# Autodesk Inventor assembly: FirstIntakes
(part 2 of 3)
- [Mate]: 1_2” Hex Bore Plastic VersaHub v2 (217-8079):20 ↔ #8-32 Nylock Nut (275-1027):49
- [Angle] (0 deg): 1_2” Hex Bore Plastic VersaHub v2 (217-8079):20 ↔ #8-32 Nylock Nut (275-1027):54
- [Angle] (0 deg): 1_2” Hex Bore Plastic VersaHub v2 (217-8079):20 ↔ #8-32 Nylock Nut (275-1027):49
- [Angle] (0 deg): 1_2” Hex Bore Plastic VersaHub v2 (217-8079):20 ↔ #8-32 Nylock Nut (275-1027):53
- [Angle] (0 deg): 1_2” Hex Bore Plastic VersaHub v2 (217-8079):20 ↔ #8-32 Nylock Nut (275-1027):50
- [Angle] (0 deg): 1_2” Hex Bore Plastic VersaHub v2 (217-8079):20 ↔ #8-32 Nylock Nut (275-1027):52
- [Angle] (0 deg): 1_2” Hex Bore Plastic VersaHub v2 (217-8079):20 ↔ #8-32 Nylock Nut (275-1027):51
- [Mate]: 1_2” Hex Bore Plastic VersaHub v2 (217-8079):19 ↔ 1_4 Acetal Spacer - 1_2 Hex (217-2758):10
- [Angle] (0 deg): 1_2” Hex Bore Plastic VersaHub v2 (217-8079):19 ↔ 1_4 Acetal Spacer - 1_2 Hex (217-2758):10
- [Mate]: 1_2” Hex Bore Plastic VersaHub v2 (217-8079):19 ↔ 1_4 Acetal Spacer - 1_2 Hex (217-2758):10
- Mate:406: 5 Straight Flex Wheel (60A) (217-6455):4 ↔ 5 Straight Flex Wheel (60A) (217-6455):10
- Mate:407: 5 Straight Flex Wheel (60A) (217-6455):4 ↔ 5 Straight Flex Wheel (60A) (217-6455):11
- Mate:410: 5 Straight Flex Wheel (60A) (217-6455):5 ↔ 5 Straight Flex Wheel (60A) (217-6455):6
- [Mate]: 5 Straight Flex Wheel (60A) (217-6455):12 ↔ 1_2” Hex Bore Plastic VersaHub v2 (217-8079):22
- [Mate]: 5 Straight Flex Wheel (60A) (217-6455):12 ↔ 1_2” Hex Bore Plastic VersaHub v2 (217-8079):22
- [Mate]: 5 Straight Flex Wheel (60A) (217-6455):12 ↔ 1_2” Hex Bore Plastic VersaHub v2 (217-8079):22
- [Mate]: 5 Straight Flex Wheel (60A) (217-6455):12 ↔ 1_2” Hex Bore Plastic VersaHub v2 (217-8079):21
- [Mate]: 5 Straight Flex Wheel (60A) (217-6455):12 ↔ 1_2” Hex Bore Plastic VersaHub v2 (217-8079):21
- [Mate]: 5 Straight Flex Wheel (60A) (217-6455):12 ↔ 1_2” Hex Bore Plastic VersaHub v2 (217-8079):21
- [Mate]: 1_2” Hex Bore Plastic VersaHub v2 (217-8079):21 ↔ #8-32 x 2.000 Star Drive Screw (276-8015):57
- [Mate]: 1_2” Hex Bore Plastic VersaHub v2 (217-8079):21 ↔ #8-32 x 2.000 Star Drive Screw (276-8015):58
- [Mate]: 1_2” Hex Bore Plastic VersaHub v2 (217-8079):21 ↔ #8-32 x 2.000 Star Drive Screw (276-8015):60
- [Mate]: 1_2” Hex Bore Plastic VersaHub v2 (217-8079):21 ↔ #8-32 x 2.000 Star Drive Screw (276-8015):55
- [Mate]: 1_2” Hex Bore Plastic VersaHub v2 (217-8079):21 ↔ #8-32 x 2.000 Star Drive Screw (276-8015):56
- [Mate]: 1_2” Hex Bore Plastic VersaHub v2 (217-8079):21 ↔ #8-32 x 2.000 Star Drive Screw (276-8015):59
- [Mate]: 1_2” Hex Bore Plastic VersaHub v2 (217-8079):21 ↔ #8-32 x 2.000 Star Drive Screw (276-8015):56
- [Mate]: 1_2” Hex Bore Plastic VersaHub v2 (217-8079):21 ↔ #8-32 x 2.000 Star Drive Screw (276-8015):58
- [Mate]: 1_2” Hex Bore Plastic VersaHub v2 (217-8079):21 ↔ #8-32 x 2.000 Star Drive Screw (276-8015):57
- [Mate]: 1_2” Hex Bore Plastic VersaHub v2 (217-8079):21 ↔ #8-32 x 2.000 Star Drive Screw (276-8015):59
- [Mate]: 1_2” Hex Bore Plastic VersaHub v2 (217-8079):21 ↔ #8-32 x 2.000 Star Drive Screw (276-8015):55
- [Mate]: 1_2” Hex Bore Plastic VersaHub v2 (217-8079):21 ↔ #8-32 x 2.000 Star Drive Screw (276-8015):60
- [Mate]: #8-32 x 2.000 Star Drive Screw (276-8015):57 ↔ #8-32 Nylock Nut (275-1027):60
- [Mate]: #8-32 x 2.000 Star Drive Screw (276-8015):60 ↔ #8-32 Nylock Nut (275-1027):55
- [Mate]: #8-32 x 2.000 Star Drive Screw (276-8015):55 ↔ #8-32 Nylock Nut (275-1027):59
- [Mate]: #8-32 x 2.000 Star Drive Screw (276-8015):59 ↔ #8-32 Nylock Nut (275-1027):56
- [Mate]: #8-32 x 2.000 Star Drive Screw (276-8015):56 ↔ #8-32 Nylock Nut (275-1027):58
- [Mate]: #8-32 x 2.000 Star Drive Screw (276-8015):58 ↔ #8-32 Nylock Nut (275-1027):57
- [Mate]: 1_2” Hex Bore Plastic VersaHub v2 (217-8079):22 ↔ #8-32 Nylock Nut (275-1027):60
- [Mate]: 1_2” Hex Bore Plastic VersaHub v2 (217-8079):22 ↔ #8-32 Nylock Nut (275-1027):57
- [Mate]: 1_2” Hex Bore Plastic VersaHub v2 (217-8079):22 ↔ #8-32 Nylock Nut (275-1027):58
- [Mate]: 1_2” Hex Bore Plastic VersaHub v2 (217-8079):22 ↔ #8-32 Nylock Nut (275-1027):56
- [Mate]: 1_2” Hex Bore Plastic VersaHub v2 (217-8079):22 ↔ #8-32 Nylock Nut (275-1027):59
- [Mate]: 1_2” Hex Bore Plastic VersaHub v2 (217-8079):22 ↔ #8-32 Nylock Nut (275-1027):55
- [Angle] (0 deg): 1_2” Hex Bore Plastic VersaHub v2 (217-8079):22 ↔ #8-32 Nylock Nut (275-1027):60
- [Angle] (0 deg): 1_2” Hex Bore Plastic VersaHub v2 (217-8079):22 ↔ #8-32 Nylock Nut (275-1027):55
- [Angle] (0 deg): 1_2” Hex Bore Plastic VersaHub v2 (217-8079):22 ↔ #8-32 Nylock Nut (275-1027):59
- [Angle] (0 deg): 1_2” Hex Bore Plastic VersaHub v2 (217-8079):22 ↔ #8-32 Nylock Nut (275-1027):56
- [Angle] (0 deg): 1_2” Hex Bore Plastic VersaHub v2 (217-8079):22 ↔ #8-32 Nylock Nut (275-1027):58
- [Angle] (0 deg): 1_2” Hex Bore Plastic VersaHub v2 (217-8079):22 ↔ #8-32 Nylock Nut (275-1027):57
- Mate:444: 5 Straight Flex Wheel (60A) (217-6455):5 ↔ 5 Straight Flex Wheel (60A) (217-6455):12
- Mate:446: 1_2” Hex Bore Plastic VersaHub v2 (217-8079):22 ↔ 1_2 Acetal Spacer - 1_2 Hex (217-2758):3
- Angle:132 (0 deg): 1_2” Hex Bore Plastic VersaHub v2 (217-8079):22 ↔ 1_2 Acetal Spacer - 1_2 Hex (217-2758):3
- Mate:447: 1_2” Hex Bore Plastic VersaHub v2 (217-8079):22 ↔ 1_2 Acetal Spacer - 1_2 Hex (217-2758):3
- Flush:1: 5 Straight Flex Wheel (60A) (217-6455):4 ↔ 5 Straight Flex Wheel (60A) (217-6455):5
- Flush:2: 5 Straight Flex Wheel (60A) (217-6455):3 ↔ 5 Straight Flex Wheel (60A) (217-6455):4
- Mate:448: 13.75mm (1_2 ThunderHex ID) x 1.125 OD x 0.313 WD (Flanged Bearing) (217-4006):2 ↔ 5 Straight Flex Wheel (60A) (217-6455):4
- Angle:133 (0 deg): 1 x 1 x 0.040 x 14 Intake Pre-Drilled VersaFrame Aluminum Tube Stock Cut Modified (217-3426):1 ↔ 24T x 9mm Wide Double Flange Aluminum Pulley (HTD 5mm, 1_2” Hex Bore) (217-3227):8
- Angle:134 (0 deg): 1 x 1 x 0.040 x 14 Intake Pre-Drilled VersaFrame Aluminum Tube Stock Cut Modified (217-3426):1 ↔ 24T x 9mm Wide Double Flange Aluminum Pulley (HTD 5mm, 1_2” Hex Bore) (217-3227):6
- Angle:135 (0 deg): 1 x 1 x 0.040 x 14 Intake Pre-Drilled VersaFrame Aluminum Tube Stock Cut Modified (217-3426):1 ↔ 1_4 Acetal Spacer - 1_2 Hex (217-2758):13
- Angle:136 (0 deg): 1 x 1 x 0.040 x 14 Intake Pre-Drilled VersaFrame Aluminum Tube Stock Cut Modified (217-3426):1 ↔ 1_2” Hex Bore Plastic VersaHub v2 (217-8079):20
- Angle:139 (0 deg): 24T x 9mm Wide Double Flange Aluminum Pulley (HTD 5mm, 1_2” Hex Bore) (217-3227):8 ↔ 1_2 Acetal Spacer - 1_2 Hex (217-2758):3
- Angle:140 (0 deg): 24T x 9mm Wide Double Flange Aluminum Pulley (HTD 5mm, 1_2” Hex Bore) (217-3227):8 ↔ 1_2 Acetal Spacer - 1_2 Hex (217-2758):3
- Flush:4: 5 Straight Flex Wheel (60A) (217-6455):6 ↔ 5 Straight Flex Wheel (60A) (217-6455):11
- Mate:452: 24T x 9mm Wide Double Flange Aluminum Pulley (HTD 5mm, 1_2” Hex Bore) (217-3227):6 ↔ 1_4 Acetal Spacer - 1_2 Hex (217-2758):10
- Mate:453: 5 Straight Flex Wheel (60A) (217-6455):11 ↔ 80T x 9mm Wide Timing Belt (HTD 5mm)(217-3456):2
- Mate:454: 5 Straight Flex Wheel (60A) (217-6455):11 ↔ 80T x 9mm Wide Timing Belt (HTD 5mm)(217-3456):1
- Mate:455: 5 Straight Flex Wheel (60A) (217-6455):3 ↔ 80T x 9mm Wide Timing Belt (HTD 5mm)(217-3456):2
- Mate:456: 5 Straight Flex Wheel (60A) (217-6455):6 ↔ 80T x 9mm Wide Timing Belt (HTD 5mm)(217-3456):1
- Flush:5: 24T x 9mm Wide Double Flange Aluminum Pulley (HTD 5mm, 1_2” Hex Bore) (217-3227):3 ↔ 80T x 9mm Wide Timing Belt (HTD 5mm)(217-3456):2
- Flush:6: 24T x 9mm Wide Double Flange Aluminum Pulley (HTD 5mm, 1_2” Hex Bore) (217-3227):6 ↔ 80T x 9mm Wide Timing Belt (HTD 5mm)(217-3456):1
- Mate:462: 1_2” Hex Bore Plastic VersaHub v2 (217-8079):17 ↔ Clamping Shaft Collar - 1_2 Hex ID (217-2737):4
- Angle:181 (0 deg): 1_2” Hex Bore Plastic VersaHub v2 (217-8079):17 ↔ Clamping Shaft Collar - 1_2 Hex ID (217-2737):4
- Angle:182 (0 deg): Clamping Shaft Collar - 1_2 Hex ID (217-2737):4 ↔ Clamping Shaft Collar - 1_2 Hex ID (217-2737):6
- Mate:463: 1_4 Acetal Spacer - 1_2 Hex (217-2758):12 ↔ Clamping Shaft Collar - 1_2 Hex ID (217-2737):6
- Mate:464: 1_2” Hex Bore Plastic VersaHub v2 (217-8079):20 ↔ Clamping Shaft Collar - 1_2 Hex ID (217-2737):3
- Mate:465: 1_2” Hex Bore Plastic VersaHub v2 (217-8079):20 ↔ Clamping Shaft Collar - 1_2 Hex ID (217-2737):3
- Angle:183 (0 deg): 1_2” Hex Bore Plastic VersaHub v2 (217-8079):20 ↔ Clamping Shaft Collar - 1_2 Hex ID (217-2737):3
- Angle:185 (0 deg): 1_2” Hex Bore Plastic VersaHub v2 (217-8079):4 ↔ Clamping Shaft Collar - 1_2 Hex ID (217-2737):9
- Angle:186 (0 deg): 1_2” Hex Bore Plastic VersaHub v2 (217-8079):4 ↔ Clamping Shaft Collar - 1_2 Hex ID (217-2737):9
- Mate:467: 1_2” Hex Bore Plastic VersaHub v2 (217-8079):4 ↔ Clamping Shaft Collar - 1_2 Hex ID (217-2737):9
- Mate:468: 1_2” Hex Bore Plastic VersaHub v2 (217-8079):4 ↔ Clamping Shaft Collar - 1_2 Hex ID (217-2737):9
- Mate:470: 24T x 9mm Wide Double Flange Aluminum Pulley (HTD 5mm, 1_2” Hex Bore) (217-3227):3 ↔ Clamping Shaft Collar - 1_2 Hex ID (217-2737):7
- Mate:471: 24T x 9mm Wide Double Flange Aluminum Pulley (HTD 5mm, 1_2” Hex Bore) (217-3227):3 ↔ Clamping Shaft Collar - 1_2 Hex ID (217-2737):10
- Mate:472: 24T x 9mm Wide Double Flange Aluminum Pulley (HTD 5mm, 1_2” Hex Bore) (217-3227):3 ↔ Clamping Shaft Collar - 1_2 Hex ID (217-2737):10
- Angle:188 (0 deg): 24T x 9mm Wide Double Flange Aluminum Pulley (HTD 5mm, 1_2” Hex Bore) (217-3227):3 ↔ Clamping Shaft Collar - 1_2 Hex ID (217-2737):10
- Angle:189 (0 deg): Clamping Shaft Collar - 1_2 Hex ID (217-2737):7 ↔ Clamping Shaft Collar - 1_2 Hex ID (217-2737):10
- Mate:474: 1_2” Hex Bore Plastic VersaHub v2 (217-8079):17 ↔ 1_4 Acetal Spacer - 1_2 Hex (217-2758):13
- Mate:475: 1_2” Hex Bore Plastic VersaHub v2 (217-8079):18 ↔ Clamping Shaft Collar - 1_2 Hex ID (217-2737):4
- Flush:11: 5 Straight Flex Wheel (60A) (217-6455):10 ↔ 5 Straight Flex Wheel (60A) (217-6455):12
- Mate:476: 24T x 9mm Wide Double Flange Aluminum Pulley (HTD 5mm, 1_2” Hex Bore) (217-3227):5 ↔ 1_4 Acetal Spacer - 1_2 Hex (217-2758):13
- Mate:477: 5 Straight Flex Wheel (60A) (217-6455):4 ↔ 5 Straight Flex Wheel (60A) (217-6455):10
- Mate:486: 1_2 Acetal Spacer - 1_2 Hex (217-2758):3 ↔ 1_16 Acetal Spacer - 1_2 Hex (217-2758):2
- Angle:199 (0 deg): 1_2 Acetal Spacer - 1_2 Hex (217-2758):3 ↔ 1_16 Acetal Spacer - 1_2 Hex (217-2758):2
- Mate:487: 1_2 Acetal Spacer - 1_2 Hex (217-2758):4 ↔ 1_16 Acetal Spacer - 1_2 Hex (217-2758):2
- Mate:494: 1 x 1 x 0.040 x 14 Intake Pre-Drilled VersaFrame Aluminum Tube Stock Cut Modified (217-3426):1 ↔ #8-32 x 1.500 Star Drive Screw (276-4998):1
- Mate:495: 1 x 1 x 0.040 x 14 Intake Pre-Drilled VersaFrame Aluminum Tube Stock Cut Modified (217-3426):1 ↔ #8-32 x 1.500 Star Drive Screw (276-4998):2
- Mate:496: 1 x 1 x 0.040 x 14 Intake Pre-Drilled VersaFrame Aluminum Tube Stock Cut Modified (217-3426):1 ↔ #8-32 x 1.500 Star Drive Screw (276-4998):3
- Mate:497: 1 x 1 x 0.040 x 14 Intake Pre-Drilled VersaFrame Aluminum Tube Stock Cut Modified (217-3426):1 ↔ #8-32 x 1.500 Star Drive Screw (276-4998):4
- Mate:498: 1 x 1 x 0.040 x 14 Intake Pre-Drilled VersaFrame Aluminum Tube Stock Cut Modified (217-3426):1 ↔ #8-32 x 1.500 Star Drive Screw (276-4998):5
- Mate:499: 1 x 1 x 0.040 x 14 Intake Pre-Drilled VersaFrame Aluminum Tube Stock Cut Modified (217-3426):1 ↔ #8-32 x 1.500 Star Drive Screw (276-4998):7
- Mate:500: 1 x 1 x 0.040 x 14 Intake Pre-Drilled VersaFrame Aluminum Tube Stock Cut Modified (217-3426):1 ↔ #8-32 x 1.500 Star Drive Screw (276-4998):6
- Mate:501: 1 x 1 x 0.040 x 14 Intake Pre-Drilled VersaFrame Aluminum Tube Stock Cut Modified (217-3426):1 ↔ #8-32 x 1.500 Star Drive Screw (276-4998):8
- Mate:505: 1 x 1 x 0.040 x 14 Intake Pre-Drilled VersaFrame Aluminum Tube Stock Cut Modified (217-3426):1 ↔ #8-32 x 1.500 Star Drive Screw (276-4998):4
- Mate:506: 1 x 1 x 0.040 x 14 Intake Pre-Drilled VersaFrame Aluminum Tube Stock Cut Modified (217-3426):1 ↔ #8-32 x 1.500 Star Drive Screw (276-4998):5
- Mate:510: #8-32 x 1.500 Star Drive Screw (276-4998):1 ↔ #8-32 Nylock Nut (275-1027):65
- Mate:511: #8-32 x 1.500 Star Drive Screw (276-4998):2 ↔ #8-32 Nylock Nut (275-1027):63
- Mate:512: #8-32 x 1.500 Star Drive Screw (276-4998):3 ↔ #8-32 Nylock Nut (275-1027):64
- Mate:513: #8-32 x 1.500 Star Drive Screw (276-4998):5 ↔ #8-32 Nylock Nut (275-1027):62
- Mate:514: #8-32 x 1.500 Star Drive Screw (276-4998):4 ↔ #8-32 Nylock Nut (275-1027):61
- Mate:515: #8-32 x 1.500 Star Drive Screw (276-4998):8 ↔ #8-32 Nylock Nut (275-1027):66
- Mate:516: #8-32 x 1.500 Star Drive Screw (276-4998):6 ↔ #8-32 Nylock Nut (275-1027):67
- Mate:517: #8-32 x 1.500 Star Drive Screw (276-4998):7 ↔ #8-32 Nylock Nut (275-1027):68
- Mate:521: VersaFrame Side Bearing Gusset (217-3553):2 ↔ #8-32 Nylock Nut (275-1027):61
- Mate:522: VersaFrame Side Bearing Gusset (217-3553):2 ↔ #8-32 Nylock Nut (275-1027):62
- Mate:523: VersaFrame Side Bearing Gusset (217-3553):3 ↔ #8-32 Nylock Nut (275-1027):65
- Mate:524: VersaFrame Side Bearing Gusset (217-3553):3 ↔ #8-32 Nylock Nut (275-1027):63
- Mate:525: VersaFrame Side Bearing Gusset (217-3553):3 ↔ #8-32 Nylock Nut (275-1027):64
- Angle:203 (0 deg): 1 x 1 x 0.040 x 14 Intake Pre-Drilled VersaFrame Aluminum Tube Stock Cut Modified (217-3426):1 ↔ #8-32 Nylock Nut (275-1027):66
- Angle:204 (0 deg): 1 x 1 x 0.040 x 14 Intake Pre-Drilled VersaFrame Aluminum Tube Stock Cut Modified (217-3426):1 ↔ #8-32 Nylock Nut (275-1027):67
- Angle:205 (0 deg): 1 x 1 x 0.040 x 14 Intake Pre-Drilled VersaFrame Aluminum Tube Stock Cut Modified (217-3426):1 ↔ #8-32 Nylock Nut (275-1027):68
- Angle:206 (0 deg): 1 x 1 x 0.040 x 14 Intake Pre-Drilled VersaFrame Aluminum Tube Stock Cut Modified (217-3426):1 ↔ #8-32 Nylock Nut (275-1027):61
- Angle:207 (0 deg): 1 x 1 x 0.040 x 14 Intake Pre-Drilled VersaFrame Aluminum Tube Stock Cut Modified (217-3426):1 ↔ #8-32 Nylock Nut (275-1027):62
- Angle:208 (0 deg): 1 x 1 x 0.040 x 14 Intake Pre-Drilled VersaFrame Aluminum Tube Stock Cut Modified (217-3426):1 ↔ #8-32 Nylock Nut (275-1027):64
- Angle:209 (0 deg): 1 x 1 x 0.040 x 14 Intake Pre-Drilled VersaFrame Aluminum Tube Stock Cut Modified (217-3426):1 ↔ #8-32 Nylock Nut (275-1027):63
- Angle:210 (0 deg): 1 x 1 x 0.040 x 14 Intake Pre-Drilled VersaFrame Aluminum Tube Stock Cut Modified (217-3426):1 ↔ #8-32 Nylock Nut (275-1027):65
- Angle:211 (0 deg): 1 x 1 x 0.040 x 14 Intake Pre-Drilled VersaFrame Aluminum Tube Stock Cut Modified (217-3426):1 ↔ #8-32 x 1.500 Star Drive Screw (276-4998):1
- Angle:212 (0 deg): 1 x 1 x 0.040 x 14 Intake Pre-Drilled VersaFrame Aluminum Tube Stock Cut Modified (217-3426):1 ↔ #8-32 x 1.500 Star Drive Screw (276-4998):8
- Angle:213 (0 deg): 1 x 1 x 0.040 x 14 Intake Pre-Drilled VersaFrame Aluminum Tube Stock Cut Modified (217-3426):1 ↔ #8-32 x 1.500 Star Drive Screw (276-4998):7
- Angle:214 (0 deg): 1 x 1 x 0.040 x 14 Intake Pre-Drilled VersaFrame Aluminum Tube Stock Cut Modified (217-3426):1 ↔ #8-32 x 1.500 Star Drive Screw (276-4998):6
- Angle:215 (0 deg): 1 x 1 x 0.040 x 14 Intake Pre-Drilled VersaFrame Aluminum Tube Stock Cut Modified (217-3426):1 ↔ #8-32 x 1.500 Star Drive Screw (276-4998):5
- Angle:216 (0 deg): 1 x 1 x 0.040 x 14 Intake Pre-Drilled VersaFrame Aluminum Tube Stock Cut Modified (217-3426):1 ↔ #8-32 x 1.500 Star Drive Screw (276-4998):4
- Angle:217 (0 deg): 1 x 1 x 0.040 x 14 Intake Pre-Drilled VersaFrame Aluminum Tube Stock Cut Modified (217-3426):1 ↔ #8-32 x 1.500 Star Drive Screw (276-4998):3
- Angle:218 (0 deg): 1 x 1 x 0.040 x 14 Intake Pre-Drilled VersaFrame Aluminum Tube Stock Cut Modified (217-3426):1 ↔ #8-32 x 1.500 Star Drive Screw (276-4998):2
- Mate:526: 13.75mm (1_2 ThunderHex ID) x 1.125 OD x 0.313 WD (Flanged Bearing) (217-4006):2 ↔ Clamping Shaft Collar - 1_2 Hex ID (217-2737):6
- Mate:529: #8-32 Nylock Nut (275-1027):69 ↔ #8-32 x 2.000 Star Drive Screw (276-8015):61
- Mate:530: #8-32 Nylock Nut (275-1027):70 ↔ #8-32 x 2.000 Star Drive Screw (276-8015):63
- Mate:531: #8-32 Nylock Nut (275-1027):71 ↔ #8-32 x 2.000 Star Drive Screw (276-8015):66
- Mate:532: #8-32 Nylock Nut (275-1027):72 ↔ #8-32 x 2.000 Star Drive Screw (276-8015):64
- Mate:533: #8-32 Nylock Nut (275-1027):73 ↔ #8-32 x 2.000 Star Drive Screw (276-8015):65
- Mate:534: #8-32 Nylock Nut (275-1027):80 ↔ #8-32 x 2.000 Star Drive Screw (276-8015):62
- Mate:535: #8-32 Nylock Nut (275-1027):74 ↔ #8-32 x 2.000 Star Drive Screw (276-8015):67
- Mate:536: #8-32 Nylock Nut (275-1027):75 ↔ #8-32 x 2.000 Star Drive Screw (276-8015):68
- Mate:537: #8-32 Nylock Nut (275-1027):79 ↔ #8-32 x 2.000 Star Drive Screw (276-8015):69
- Mate:538: #8-32 Nylock Nut (275-1027):76 ↔ #8-32 x 2.000 Star Drive Screw (276-8015):71
- Mate:539: #8-32 Nylock Nut (275-1027):77 ↔ #8-32 x 2.000 Star Drive Screw (276-8015):70
- Mate:540: #8-32 Nylock Nut (275-1027):78 ↔ #8-32 x 2.000 Star Drive Screw (276-8015):72
- Angle:219 (0 deg): 1_2” Hex Bore Plastic VersaHub v2 (217-8079):6 ↔ #8-32 Nylock Nut (275-1027):70
- Angle:220 (0 deg): 1_2” Hex Bore Plastic VersaHub v2 (217-8079):6 ↔ #8-32 Nylock Nut (275-1027):71
- Angle:221 (0 deg): 1_2” Hex Bore Plastic VersaHub v2 (217-8079):6 ↔ #8-32 Nylock Nut (275-1027):72
- Angle:222 (0 deg): 1_2” Hex Bore Plastic VersaHub v2 (217-8079):6 ↔ #8-32 Nylock Nut (275-1027):73
- Angle:223 (0 deg): 1_2” Hex Bore Plastic VersaHub v2 (217-8079):6 ↔ #8-32 Nylock Nut (275-1027):80
- Angle:224 (0 deg): 1_2” Hex Bore Plastic VersaHub v2 (217-8079):6 ↔ #8-32 Nylock Nut (275-1027):69
- Angle:225 (0 deg): 1_2” Hex Bore Plastic VersaHub v2 (217-8079):8 ↔ #8-32 Nylock Nut (275-1027):78
- Angle:226 (0 deg): 1_2” Hex Bore Plastic VersaHub v2 (217-8079):8 ↔ #8-32 Nylock Nut (275-1027):76
- Angle:227 (0 deg): 1_2” Hex Bore Plastic VersaHub v2 (217-8079):8 ↔ #8-32 Nylock Nut (275-1027):75
- Angle:228 (0 deg): 1_2” Hex Bore Plastic VersaHub v2 (217-8079):8 ↔ #8-32 Nylock Nut (275-1027):74
- Angle:229 (0 deg): 1_2” Hex Bore Plastic VersaHub v2 (217-8079):8 ↔ #8-32 Nylock Nut (275-1027):77
- Angle:230 (0 deg): 1_2” Hex Bore Plastic VersaHub v2 (217-8079):8 ↔ #8-32 Nylock Nut (275-1027):79
- Mate:541: 1_2” Hex Bore Plastic VersaHub v2 (217-8079):8 ↔ #8-32 Nylock Nut (275-1027):74
- Mate:542: 1_2” Hex Bore Plastic VersaHub v2 (217-8079):8 ↔ #8-32 Nylock Nut (275-1027):79
- Mate:543: 1_2” Hex Bore Plastic VersaHub v2 (217-8079):8 ↔ #8-32 Nylock Nut (275-1027):75
- Mate:544: 1_2” Hex Bore Plastic VersaHub v2 (217-8079):8 ↔ #8-32 Nylock Nut (275-1027):77
- Mate:545: 1_2” Hex Bore Plastic VersaHub v2 (217-8079):8 ↔ #8-32 Nylock Nut (275-1027):76
- Mate:546: 1_2” Hex Bore Plastic VersaHub v2 (217-8079):8 ↔ #8-32 Nylock Nut (275-1027):78
- Mate:547: 1_2” Hex Bore Plastic VersaHub v2 (217-8079):6 ↔ #8-32 Nylock Nut (275-1027):73
- Mate:548: 1_2” Hex Bore Plastic VersaHub v2 (217-8079):6 ↔ #8-32 Nylock Nut (275-1027):71
- Mate:550: 1_2” Hex Bore Plastic VersaHub v2 (217-8079):6 ↔ #8-32 Nylock Nut (275-1027):72
- Mate:551: 1_2” Hex Bore Plastic VersaHub v2 (217-8079):6 ↔ #8-32 Nylock Nut (275-1027):80
- Mate:552: 1_2” Hex Bore Plastic VersaHub v2 (217-8079):6 ↔ #8-32 Nylock Nut (275-1027):69
- Mate:553: 1_2” Hex Bore Plastic VersaHub v2 (217-8079):6 ↔ #8-32 Nylock Nut (275-1027):70
- Angle:231 (0 deg): 1_2” Hex Bore Plastic VersaHub v2 (217-8079):21 ↔ Clamping Shaft Collar - 1_2 Hex ID (217-2737):12
- Mate:554: 1_2” Hex Bore Plastic VersaHub v2 (217-8079):21 ↔ Clamping Shaft Collar - 1_2 Hex ID (217-2737):12
- Mate:555: 1_2” Hex Bore Plastic VersaHub v2 (217-8079):21 ↔ Clamping Shaft Collar - 1_2 Hex ID (217-2737):12
- Angle:232 (0 deg): 1_2” Hex Bore Plastic VersaHub v2 (217-8079):10 ↔ Clamping Shaft Collar - 1_2 Hex ID (217-2737):11
- Mate:556: 1_2” Hex Bore Plastic VersaHub v2 (217-8079):10 ↔ Clamping Shaft Collar - 1_2 Hex ID (217-2737):11
- Mate:557: 1_2” Hex Bore Plastic VersaHub v2 (217-8079):10 ↔ Clamping Shaft Collar - 1_2 Hex ID (217-2737):11
- Angle:233 (0 deg): Clamping Shaft Collar - 1_2 Hex ID (217-2737):3 ↔ Clamping Shaft Collar - 1_2 Hex ID (217-2737):11
- Mate:558: 5 Straight Flex Wheel (60A) (217-6455):3
- Flush:560: 5 Straight Flex Wheel (60A) (217-6455):3
- Flush:14: 5 Straight Flex Wheel (60A) (217-6455):3
- [Mate]: VersaFrame Side Bearing Gusset (217-3553):4 ↔ 1 x 1 x 0.040 x 14 Intake Pre-Drilled VersaFrame Aluminum Tube Stock Cut Modified (217-3426):2
- [Mate]: VersaFrame Side Bearing Gusset (217-3553):4 ↔ 1 x 1 x 0.040 x 14 Intake Pre-Drilled VersaFrame Aluminum Tube Stock Cut Modified (217-3426):2
- [Mate]: VersaFrame Side Bearing Gusset (217-3553):5 ↔ 1 x 1 x 0.040 x 14 Intake Pre-Drilled VersaFrame Aluminum Tube Stock Cut Modified (217-3426):2
- [Mate]: VersaFrame Side Bearing Gusset (217-3553):5 ↔ 1 x 1 x 0.040 x 14 Intake Pre-Drilled VersaFrame Aluminum Tube Stock Cut Modified (217-3426):2
- [Mate]: VersaFrame Side Bearing Gusset (217-3553):5 ↔ 1 x 1 x 0.040 x 14 Intake Pre-Drilled VersaFrame Aluminum Tube Stock Cut Modified (217-3426):2
- [Mate]: VersaFrame Side Bearing Gusset (217-3553):4 ↔ 13.75mm (1_2 ThunderHex ID) x 1.125 OD x 0.313 WD (Flanged Bearing) (217-4006):6
- [Mate]: VersaFrame Side Bearing Gusset (217-3553):5 ↔ 13.75mm (1_2 ThunderHex ID) x 1.125 OD x 0.313 WD (Flanged Bearing) (217-4006):5
- [Mate]: VersaFrame Side Bearing Gusset (217-3553):5 ↔ 13.75mm (1_2 ThunderHex ID) x 1.125 OD x 0.313 WD (Flanged Bearing) (217-4006):5
- [Mate]: VersaFrame Side Bearing Gusset (217-3553):4 ↔ 13.75mm (1_2 ThunderHex ID) x 1.125 OD x 0.313 WD (Flanged Bearing) (217-4006):6
- [Angle] (0 deg): 1 x 1 x 0.040 x 14 Intake Pre-Drilled VersaFrame Aluminum Tube Stock Cut Modified (217-3426):2 ↔ 13.75mm (1_2 ThunderHex ID) x 1.125 OD x 0.313 WD (Flanged Bearing) (217-4006):5
- [Angle] (0 deg): 1 x 1 x 0.040 x 14 Intake Pre-Drilled VersaFrame Aluminum Tube Stock Cut Modified (217-3426):2 ↔ 13.75mm (1_2 ThunderHex ID) x 1.125 OD x 0.313 WD (Flanged Bearing) (217-4006):6
- [Mate]: 1 x 1 x 0.040 x 14 Intake Pre-Drilled VersaFrame Aluminum Tube Stock Cut Modified (217-3426):2 ↔ #8-32 x 1.500 Star Drive Screw (276-4998):9
- [Mate]: 1 x 1 x 0.040 x 14 Intake Pre-Drilled VersaFrame Aluminum Tube Stock Cut Modified (217-3426):2 ↔ #8-32 x 1.500 Star Drive Screw (276-4998):10
- [Mate]: 1 x 1 x 0.040 x 14 Intake Pre-Drilled VersaFrame Aluminum Tube Stock Cut Modified (217-3426):2 ↔ #8-32 x 1.500 Star Drive Screw (276-4998):11
- [Mate]: 1 x 1 x 0.040 x 14 Intake Pre-Drilled VersaFrame Aluminum Tube Stock Cut Modified (217-3426):2 ↔ #8-32 x 1.500 Star Drive Screw (276-4998):12
- [Mate]: 1 x 1 x 0.040 x 14 Intake Pre-Drilled VersaFrame Aluminum Tube Stock Cut Modified (217-3426):2 ↔ #8-32 x 1.500 Star Drive Screw (276-4998):13
- [Mate]: 1 x 1 x 0.040 x 14 Intake Pre-Drilled VersaFrame Aluminum Tube Stock Cut Modified (217-3426):2 ↔ #8-32 x 1.500 Star Drive Screw (276-4998):15
- [Mate]: 1 x 1 x 0.040 x 14 Intake Pre-Drilled VersaFrame Aluminum Tube Stock Cut Modified (217-3426):2 ↔ #8-32 x 1.500 Star Drive Screw (276-4998):14
- [Mate]: 1 x 1 x 0.040 x 14 Intake Pre-Drilled VersaFrame Aluminum Tube Stock Cut Modified (217-3426):2 ↔ #8-32 x 1.500 Star Drive Screw (276-4998):16
- Mate:583: Intake Joint Holder Using 1__16 Gray Tinted Polycarbonate Sheet (36 x 72) (217-6627):1 ↔ #8-32 x 1.500 Star Drive Screw (276-4998):16
- Mate:584: Intake Joint Holder Using 1__16 Gray Tinted Polycarbonate Sheet (36 x 72) (217-6627):1 ↔ #8-32 x 1.500 Star Drive Screw (276-4998):14
- Mate:585: Intake Joint Holder Using 1__16 Gray Tinted Polycarbonate Sheet (36 x 72) (217-6627):1 ↔ #8-32 x 1.500 Star Drive Screw (276-4998):15
- [Mate]: 1 x 1 x 0.040 x 14 Intake Pre-Drilled VersaFrame Aluminum Tube Stock Cut Modified (217-3426):2 ↔ #8-32 x 1.500 Star Drive Screw (276-4998):12
- [Mate]: 1 x 1 x 0.040 x 14 Intake Pre-Drilled VersaFrame Aluminum Tube Stock Cut Modified (217-3426):2 ↔ #8-32 x 1.500 Star Drive Screw (276-4998):13
- [Mate]: 1 x 1 x 0.040 x 14 Intake Pre-Drilled VersaFrame Aluminum Tube Stock Cut Modified (217-3426):2 ↔ #8-32 x 1.500 Star Drive Screw (276-4998):10
- Mate:590: Intake VersaFrame VersaPlanetary Side Mount Modified (217-4239):1 ↔ #8-32 x 1.500 Star Drive Screw (276-4998):9
- [Mate]: #8-32 x 1.500 Star Drive Screw (276-4998):9 ↔ #8-32 Nylock Nut (275-1027):85
- [Mate]: #8-32 x 1.500 Star Drive Screw (276-4998):10 ↔ #8-32 Nylock Nut (275-1027):83
- [Mate]: #8-32 x 1.500 Star Drive Screw (276-4998):11 ↔ #8-32 Nylock Nut (275-1027):84
- [Mate]: #8-32 x 1.500 Star Drive Screw (276-4998):13 ↔ #8-32 Nylock Nut (275-1027):82
- [Mate]: #8-32 x 1.500 Star Drive Screw (276-4998):12 ↔ #8-32 Nylock Nut (275-1027):81
- [Mate]: #8-32 x 1.500 Star Drive Screw (276-4998):16 ↔ #8-32 Nylock Nut (275-1027):86
- [Mate]: #8-32 x 1.500 Star Drive Screw (276-4998):14 ↔ #8-32 Nylock Nut (275-1027):87
- [Mate]: #8-32 x 1.500 Star Drive Screw (276-4998):15 ↔ #8-32 Nylock Nut (275-1027):88
- [Mate]: VersaFrame Side Bearing Gusset (217-3553):4 ↔ #8-32 Nylock Nut (275-1027):88
- [Mate]: VersaFrame Side Bearing Gusset (217-3553):4 ↔ #8-32 Nylock Nut (275-1027):87
- [Mate]: VersaFrame Side Bearing Gusset (217-3553):5 ↔ #8-32 Nylock Nut (275-1027):81
- [Mate]: VersaFrame Side Bearing Gusset (217-3553):5 ↔ #8-32 Nylock Nut (275-1027):82
- [Angle] (0 deg): 1 x 1 x 0.040 x 14 Intake Pre-Drilled VersaFrame Aluminum Tube Stock Cut Modified (217-3426):2 ↔ #8-32 Nylock Nut (275-1027):86
- [Angle] (0 deg): 1 x 1 x 0.040 x 14 Intake Pre-Drilled VersaFrame Aluminum Tube Stock Cut Modified (217-3426):2 ↔ #8-32 Nylock Nut (275-1027):87
- [Angle] (0 deg): 1 x 1 x 0.040 x 14 Intake Pre-Drilled VersaFrame Aluminum Tube Stock Cut Modified (217-3426):2 ↔ #8-32 Nylock Nut (275-1027):88
- [Angle] (0 deg): 1 x 1 x 0.040 x 14 Intake Pre-Drilled VersaFrame Aluminum Tube Stock Cut Modified (217-3426):2 ↔ #8-32 Nylock Nut (275-1027):81
- [Angle] (0 deg): 1 x 1 x 0.040 x 14 Intake Pre-Drilled VersaFrame Aluminum Tube Stock Cut Modified (217-3426):2 ↔ #8-32 Nylock Nut (275-1027):82
- [Angle] (0 deg): 1 x 1 x 0.040 x 14 Intake Pre-Drilled VersaFrame Aluminum Tube Stock Cut Modified (217-3426):2 ↔ #8-32 Nylock Nut (275-1027):84
- [Angle] (0 deg): 1 x 1 x 0.040 x 14 Intake Pre-Drilled VersaFrame Aluminum Tube Stock Cut Modified (217-3426):2 ↔ #8-32 Nylock Nut (275-1027):83
- [Angle] (0 deg): 1 x 1 x 0.040 x 14 Intake Pre-Drilled VersaFrame Aluminum Tube Stock Cut Modified (217-3426):2 ↔ #8-32 Nylock Nut (275-1027):85
- [Angle] (0 deg): 1 x 1 x 0.040 x 14 Intake Pre-Drilled VersaFrame Aluminum Tube Stock Cut Modified (217-3426):2 ↔ #8-32 x 1.500 Star Drive Screw (276-4998):9
- [Angle] (0 deg): 1 x 1 x 0.040 x 14 Intake Pre-Drilled VersaFrame Aluminum Tube Stock Cut Modified (217-3426):2 ↔ #8-32 x 1.500 Star Drive Screw (276-4998):16
- [Angle] (0 deg): 1 x 1 x 0.040 x 14 Intake Pre-Drilled VersaFrame Aluminum Tube Stock Cut Modified (217-3426):2 ↔ #8-32 x 1.500 Star Drive Screw (276-4998):15
- [Angle] (0 deg): 1 x 1 x 0.040 x 14 Intake Pre-Drilled VersaFrame Aluminum Tube Stock Cut Modified (217-3426):2 ↔ #8-32 x 1.500 Star Drive Screw (276-4998):14
- [Angle] (0 deg): 1 x 1 x 0.040 x 14 Intake Pre-Drilled VersaFrame Aluminum Tube Stock Cut Modified (217-3426):2 ↔ #8-32 x 1.500 Star Drive Screw (276-4998):13
- [Angle] (0 deg): 1 x 1 x 0.040 x 14 Intake Pre-Drilled VersaFrame Aluminum Tube Stock Cut Modified (217-3426):2 ↔ #8-32 x 1.500 Star Drive Screw (276-4998):12
- [Angle] (0 deg): 1 x 1 x 0.040 x 14 Intake Pre-Drilled VersaFrame Aluminum Tube Stock Cut Modified (217-3426):2 ↔ #8-32 x 1.500 Star Drive Screw (276-4998):11
- [Angle] (0 deg): 1 x 1 x 0.040 x 14 Intake Pre-Drilled VersaFrame Aluminum Tube Stock Cut Modified (217-3426):2 ↔ #8-32 x 1.500 Star Drive Screw (276-4998):10
- [Mate]: 13.75mm (1_2 ThunderHex ID) x 1.125 OD x 0.313 WD (Flanged Bearing) (217-4006):5 ↔ Clamping Shaft Collar - 1_2 Hex ID (217-2737):14
- [Mate]: VersaFrame Side Bearing Gusset (217-3553):4 ↔ #8-32 Nylock Nut (275-1027):86
- Mate:610: 5 Straight Flex Wheel (60A) (217-6455):3 ↔ 13.75mm (1_2 ThunderHex ID) x 1.125 OD x 0.313 WD (Flanged Bearing) (217-4006):6
- Mate:611: 13.75mm (1_2 ThunderHex ID) x 1.125 OD x 0.313 WD (Flanged Bearing) (217-4006):6 ↔ Clamping Shaft Collar - 1_2 Hex ID (217-2737):15
- Angle:255 (0 deg): 1 x 1 x 0.040 x 14 Intake Pre-Drilled VersaFrame Aluminum Tube Stock Cut Modified (217-3426):2 ↔ Clamping Shaft Collar - 1_2 Hex ID (217-2737):15
- Angle:257 (0 deg): 1 x 1 x 0.040 x 14 Intake Pre-Drilled VersaFrame Aluminum Tube Stock Cut Modified (217-3426):2 ↔ Clamping Shaft Collar - 1_2 Hex ID (217-2737):14
- Angle:258 (0 deg): 1 x 1 x 0.040 x 14 Intake Pre-Drilled VersaFrame Aluminum Tube Stock Cut Modified (217-3426):1 ↔ Clamping Shaft Collar - 1_2 Hex ID (217-2737):1
- Mate:614: 1 x 1 x 0.040 x 14 Intake Pre-Drilled VersaFrame Aluminum Tube Stock Cut Modified (217-3426):2 ↔ Intake Joint Holder Using 1__16 Gray Tinted Polycarbonate Sheet (36 x 72) (217-6627):1
- Mate:615: 1 x 1 x 0.040 x 14 Intake Pre-Drilled VersaFrame Aluminum Tube Stock Cut Modified (217-3426):2 ↔ Intake Joint Holder Using 1__16 Gray Tinted Polycarbonate Sheet (36 x 72) (217-6627):1
- Mate:616: 1 x 1 x 0.040 x 14 Intake Pre-Drilled VersaFrame Aluminum Tube Stock Cut Modified (217-3426):2 ↔ Intake Joint Holder Using 1__16 Gray Tinted Polycarbonate Sheet (36 x 72) (217-6627):1
- Mate:617: 13.75mm (1_2 ThunderHex ID) x 1.125 OD x 0.313 WD (Flanged Bearing) (217-4006):6 ↔ Clamping Shaft Collar - 1_2 Hex ID (217-2737):15
- Mate:618: 1 x 1 x 0.040 x 14 Intake Pre-Drilled VersaFrame Aluminum Tube Stock Cut Modified (217-3426):2 ↔ Intake Joint Holder Using 1__16 Gray Tinted Polycarbonate Sheet (36 x 72) (217-6627):2
- Mate:619: 1 x 1 x 0.040 x 14 Intake Pre-Drilled VersaFrame Aluminum Tube Stock Cut Modified (217-3426):2 ↔ Intake Joint Holder Using 1__16 Gray Tinted Polycarbonate Sheet (36 x 72) (217-6627):2
- Mate:620: 1 x 1 x 0.040 x 14 Intake Pre-Drilled VersaFrame Aluminum Tube Stock Cut Modified (217-3426):2 ↔ Intake Joint Holder Using 1__16 Gray Tinted Polycarbonate Sheet (36 x 72) (217-6627):2
- Mate:621: VersaFrame Side Bearing Gusset (217-3553):4 ↔ Intake Joint Holder Using 1__16 Gray Tinted Polycarbonate Sheet (36 x 72) (217-6627):2
- Mate:622: Intake Joint Holder Using 1__16 Gray Tinted Polycarbonate Sheet (36 x 72) (217-6627):1 ↔ 1.00 Standoff (275-1016):1
- Mate:623: Intake Joint Holder Using 1__16 Gray Tinted Polycarbonate Sheet (36 x 72) (217-6627):1 ↔ 1.00 Standoff (275-1016):1
- Mate:624: 1.00 Standoff (275-1016):1 ↔ #8-32 x 0.500 Star Drive Screw (276-4992):1
- Mate:625: Intake Joint Holder Using 1__16 Gray Tinted Polycarbonate Sheet (36 x 72) (217-6627):2 ↔ #8-32 x 0.500 Star Drive Screw (276-4992):1
- Mate:626: Intake Joint Holder Using 1__16 Gray Tinted Polycarbonate Sheet (36 x 72) (217-6627):1 ↔ #8-32 x 0.500 Star Drive Screw (276-4992):2
- Mate:627: Intake Joint Holder Using 1__16 Gray Tinted Polycarbonate Sheet (36 x 72) (217-6627):1 ↔ #8-32 x 0.500 Star Drive Screw (276-4992):2
- Mate:628: 13.75mm (1_2 ThunderHex ID) x 1.125 OD x 0.313 WD (Flanged Bearing) (217-4006):5 ↔ Clamping Shaft Collar - 1_2 Hex ID (217-2737):14
- Angle:259 (0 deg): 1 x 1 x 0.040 x 14 Intake Pre-Drilled VersaFrame Aluminum Tube Stock Cut Modified (217-3426):2 ↔ #8-32 x 0.500 Star Drive Screw (276-4992):2
- Angle:260 (0 deg): 1 x 1 x 0.040 x 14 Intake Pre-Drilled VersaFrame Aluminum Tube Stock Cut Modified (217-3426):2 ↔ #8-32 x 0.500 Star Drive Screw (276-4992):1
- Angle:261 (0 deg): 1 x 1 x 0.040 x 14 Intake Pre-Drilled VersaFrame Aluminum Tube Stock Cut Modified (217-3426):2 ↔ 1.00 Standoff (275-1016):1
- Mate:629: 13.75mm (1_2 ThunderHex ID) x 1.125 OD x 0.313 WD (Flanged Bearing) (217-4006):1 ↔ Clamping Shaft Collar - 1_2 Hex ID (217-2737):7
- Mate:630: 1 x 1 x 0.040 x 14 Intake Pre-Drilled VersaFrame Aluminum Tube Stock Cut Modified (217-3426):1 ↔ Intake Joint Holder Using 1__16 Gray Tinted Polycarbonate Sheet (36 x 72) (217-6627):3
- Mate:631: 1 x 1 x 0.040 x 14 Intake Pre-Drilled VersaFrame Aluminum Tube Stock Cut Modified (217-3426):1 ↔ Intake Joint Holder Using 1__16 Gray Tinted Polycarbonate Sheet (36 x 72) (217-6627):3
- Mate:632: 1 x 1 x 0.040 x 14 Intake Pre-Drilled VersaFrame Aluminum Tube Stock Cut Modified (217-3426):1 ↔ Intake Joint Holder Using 1__16 Gray Tinted Polycarbonate Sheet (36 x 72) (217-6627):3
- Mate:633: 1 x 1 x 0.040 x 14 Intake Pre-Drilled VersaFrame Aluminum Tube Stock Cut Modified (217-3426):1 ↔ Intake Joint Holder Using 1__16 Gray Tinted Polycarbonate Sheet (36 x 72) (217-6627):4
- Mate:634: 1 x 1 x 0.040 x 14 Intake Pre-Drilled VersaFrame Aluminum Tube Stock Cut Modified (217-3426):1 ↔ Intake Joint Holder Using 1__16 Gray Tinted Polycarbonate Sheet (36 x 72) (217-6627):4
- Mate:635: 1 x 1 x 0.040 x 14 Intake Pre-Drilled VersaFrame Aluminum Tube Stock Cut Modified (217-3426):1 ↔ Intake Joint Holder Using 1__16 Gray Tinted Polycarbonate Sheet (36 x 72) (217-6627):4
- Mate:636: VersaFrame Side Bearing Gusset (217-3553):3 ↔ Intake Joint Holder Using 1__16 Gray Tinted Polycarbonate Sheet (36 x 72) (217-6627):3
- Mate:637: Intake Joint Holder Using 1__16 Gray Tinted Polycarbonate Sheet (36 x 72) (217-6627):4 ↔ #8-32 x 1.500 Star Drive Screw (276-4998):1
- Mate:638: Intake Joint Holder Using 1__16 Gray Tinted Polycarbonate Sheet (36 x 72) (217-6627):4 ↔ #8-32 x 1.500 Star Drive Screw (276-4998):2
- Mate:639: Intake Joint Holder Using 1__16 Gray Tinted Polycarbonate Sheet (36 x 72) (217-6627):4 ↔ #8-32 x 1.500 Star Drive Screw (276-4998):3
- [Mate]: 1.00 Standoff (275-1016):2 ↔ #8-32 x 0.500 Star Drive Screw (276-4992):3
- Mate:641: Intake Joint Holder Using 1__16 Gray Tinted Polycarbonate Sheet (36 x 72) (217-6627):3 ↔ #8-32 x 0.500 Star Drive Screw (276-4992):4
- Mate:642: Intake Joint Holder Using 1__16 Gray Tinted Polycarbonate Sheet (36 x 72) (217-6627):4 ↔ #8-32 x 0.500 Star Drive Screw (276-4992):3
- Mate:643: Intake Joint Holder Using 1__16 Gray Tinted Polycarbonate Sheet (36 x 72) (217-6627):3 ↔ 1.00 Standoff (275-1016):2
- Mate:644: Intake Joint Holder Using 1__16 Gray Tinted Polycarbonate Sheet (36 x 72) (217-6627):4 ↔ #8-32 x 0.500 Star Drive Screw (276-4992):3
- Mate:645: Intake Joint Holder Using 1__16 Gray Tinted Polycarbonate Sheet (36 x 72) (217-6627):3 ↔ #8-32 x 0.500 Star Drive Screw (276-4992):4
- Angle:262 (0 deg): 1 x 1 x 0.040 x 14 Intake Pre-Drilled VersaFrame Aluminum Tube Stock Cut Modified (217-3426):1 ↔ #8-32 x 0.500 Star Drive Screw (276-4992):4
- Angle:263 (0 deg): 1 x 1 x 0.040 x 14 Intake Pre-Drilled VersaFrame Aluminum Tube Stock Cut Modified (217-3426):1 ↔ #8-32 x 0.500 Star Drive Screw (276-4992):3
- Angle:264 (0 deg): 1 x 1 x 0.040 x 14 Intake Pre-Drilled VersaFrame Aluminum Tube Stock Cut Modified (217-3426):1 ↔ 1.00 Standoff (275-1016):2
- Mate:646: Intake Joint Holder Using 1__16 Gray Tinted Polycarbonate Sheet (36 x 72) (217-6627):4 ↔ 13.75mm (1_2 ThunderHex ID) x 1.125 OD x 0.313 WD (Flanged Bearing) (217-4006):7
- Mate:647: Intake Joint Holder Using 1__16 Gray Tinted Polycarbonate Sheet (36 x 72) (217-6627):3 ↔ 13.75mm (1_2 ThunderHex ID) x 1.125 OD x 0.313 WD (Flanged Bearing) (217-4006):10
- Mate:648: Intake Joint Holder Using 1__16 Gray Tinted Polycarbonate Sheet (36 x 72) (217-6627):4 ↔ 13.75mm (1_2 ThunderHex ID) x 1.125 OD x 0.313 WD (Flanged Bearing) (217-4006):7
- Mate:649: Intake Joint Holder Using 1__16 Gray Tinted Polycarbonate Sheet (36 x 72) (217-6627):3 ↔ 13.75mm (1_2 ThunderHex ID) x 1.125 OD x 0.313 WD (Flanged Bearing) (217-4006):10
- Mate:650: Intake Joint Holder Using 1__16 Gray Tinted Polycarbonate Sheet (36 x 72) (217-6627):1 ↔ 13.75mm (1_2 ThunderHex ID) x 1.125 OD x 0.313 WD (Flanged Bearing) (217-4006):9
- Mate:651: Intake Joint Holder Using 1__16 Gray Tinted Polycarbonate Sheet (36 x 72) (217-6627):1 ↔ 13.75mm (1_2 ThunderHex ID) x 1.125 OD x 0.313 WD (Flanged Bearing) (217-4006):9
- Mate:652: Intake Joint Holder Using 1__16 Gray Tinted Polycarbonate Sheet (36 x 72) (217-6627):2 ↔ 13.75mm (1_2 ThunderHex ID) x 1.125 OD x 0.313 WD (Flanged Bearing) (217-4006):8
- Angle:265 (0 deg): 1 x 1 x 0.040 x 14 Intake Pre-Drilled VersaFrame Aluminum Tube Stock Cut Modified (217-3426):1 ↔ 13.75mm (1_2 ThunderHex ID) x 1.125 OD x 0.313 WD (Flanged Bearing) (217-4006):7
- Angle:266 (0 deg): 1 x 1 x 0.040 x 14 Intake Pre-Drilled VersaFrame Aluminum Tube Stock Cut Modified (217-3426):1 ↔ 13.75mm (1_2 ThunderHex ID) x 1.125 OD x 0.313 WD (Flanged Bearing) (217-4006):10
- Angle:267 (0 deg): 1 x 1 x 0.040 x 14 Intake Pre-Drilled VersaFrame Aluminum Tube Stock Cut Modified (217-3426):2 ↔ 13.75mm (1_2 ThunderHex ID) x 1.125 OD x 0.313 WD (Flanged Bearing) (217-4006):9
- Angle:268 (0 deg): 1 x 1 x 0.040 x 14 Intake Pre-Drilled VersaFrame Aluminum Tube Stock Cut Modified (217-3426):1 ↔ 13.75mm (1_2 ThunderHex ID) x 1.125 OD x 0.313 WD (Flanged Bearing) (217-4006):8
- Mate:653: Intake Joint Holder Using 1__16 Gray Tinted Polycarbonate Sheet (36 x 72) (217-6627):2 ↔ 13.75mm (1_2 ThunderHex ID) x 1.125 OD x 0.313 WD (Flanged Bearing) (217-4006):8
- [Mate]: 1_2 Acetal Spacer - 1_2 Hex (217-2758):5 ↔ 1_4 Acetal Spacer - 1_2 Hex (217-2758):15
- [Mate]: 1_4 Acetal Spacer - 1_2 Hex (217-2758):15 ↔ 1_8 Acetal Spacer - 1_2 Hex (217-2758):1
- [Mate]: 1_2 Acetal Spacer - 1_2 Hex (217-2758):5 ↔ 1_4 Acetal Spacer - 1_2 Hex (217-2758):15
- [Mate]: 1_4 Acetal Spacer - 1_2 Hex (217-2758):15 ↔ 1_8 Acetal Spacer - 1_2 Hex (217-2758):1
- [Angle] (0 deg): 1_2 Acetal Spacer - 1_2 Hex (217-2758):5 ↔ 1_4 Acetal Spacer - 1_2 Hex (217-2758):15
- [Angle] (0 deg): 1_2 Acetal Spacer - 1_2 Hex (217-2758):5 ↔ 1_8 Acetal Spacer - 1_2 Hex (217-2758):1
- [Mate]: 1_2 Acetal Spacer - 1_2 Hex (217-2758):6 ↔ 1_4 Acetal Spacer - 1_2 Hex (217-2758):16
- [Mate]: 1_4 Acetal Spacer - 1_2 Hex (217-2758):16 ↔ 1_8 Acetal Spacer - 1_2 Hex (217-2758):2
- [Mate]: 1_2 Acetal Spacer - 1_2 Hex (217-2758):6 ↔ 1_4 Acetal Spacer - 1_2 Hex (217-2758):16
- [Mate]: 1_4 Acetal Spacer - 1_2 Hex (217-2758):16 ↔ 1_8 Acetal Spacer - 1_2 Hex (217-2758):2
- [Angle] (0 deg): 1_2 Acetal Spacer - 1_2 Hex (217-2758):6 ↔ 1_4 Acetal Spacer - 1_2 Hex (217-2758):16
- [Angle] (0 deg): 1_2 Acetal Spacer - 1_2 Hex (217-2758):6 ↔ 1_8 Acetal Spacer - 1_2 Hex (217-2758):2
- Mate:662: 13.75mm (1_2 ThunderHex ID) x 1.125 OD x 0.313 WD (Flanged Bearing) (217-4006):9 ↔ 1_2 Acetal Spacer - 1_2 Hex (217-2758):5
- Mate:663: 13.75mm (1_2 ThunderHex ID) x 1.125 OD x 0.313 WD (Flanged Bearing) (217-4006):9 ↔ 1_2 Acetal Spacer - 1_2 Hex (217-2758):5
- Mate:664: 13.75mm (1_2 ThunderHex ID) x 1.125 OD x 0.313 WD (Flanged Bearing) (217-4006):7 ↔ 1_8 Acetal Spacer - 1_2 Hex (217-2758):2
- Mate:665: 13.75mm (1_2 ThunderHex ID) x 1.125 OD x 0.313 WD (Flanged Bearing) (217-4006):7 ↔ 1_8 Acetal Spacer - 1_2 Hex (217-2758):2
- Angle:273 (0 deg): 1 x 1 x 0.040 x 14 Intake Pre-Drilled VersaFrame Aluminum Tube Stock Cut Modified (217-3426):2 ↔ 1_2 Acetal Spacer - 1_2 Hex (217-2758):5
- Angle:274 (0 deg): 1 x 1 x 0.040 x 14 Intake Pre-Drilled VersaFrame Aluminum Tube Stock Cut Modified (217-3426):1 ↔ 1_2 Acetal Spacer - 1_2 Hex (217-2758):6
- Mate:666: 1 x 1 x 0.040 x 14 Intake Pre-Drilled VersaFrame Aluminum Tube Stock Cut Modified (217-3426):2 ↔ Intake VersaFrame VersaPlanetary Side Mount Modified (217-4239):1
- Mate:667: 1 x 1 x 0.040 x 14 Intake Pre-Drilled VersaFrame Aluminum Tube Stock Cut Modified (217-3426):2 ↔ Intake VersaFrame VersaPlanetary Side Mount Modified (217-4239):1
- Mate:668: 1 x 1 x 0.040 x 14 Intake Pre-Drilled VersaFrame Aluminum Tube Stock Cut Modified (217-3426):2 ↔ Intake VersaFrame VersaPlanetary Side Mount Modified (217-4239):1
- Mate:669: Intake VersaFrame VersaPlanetary Side Mount Modified (217-4239):1 ↔ VersaPlanetary v2 One Stage Universal Output:1
- Mate:670: Intake VersaFrame VersaPlanetary Side Mount Modified (217-4239):1 ↔ VersaPlanetary v2 One Stage Universal Output:1
- Mate:671: Intake VersaFrame VersaPlanetary Side Mount Modified (217-4239):1 ↔ VersaPlanetary v2 One Stage Universal Output:1
- Mate:673: Clamping Shaft Collar - 1_2 Hex ID (217-2737):11 ↔ VersaPlanetary v2 One Stage Universal Output:1
- Tangent:1: 24T x 9mm Wide Double Flange Aluminum Pulley (HTD 5mm, 1_2” Hex Bore) (217-3227):8 ↔ 80T x 9mm Wide Timing Belt (HTD 5mm)(217-3456):1
- Mate:674: Intake VersaFrame VersaPlanetary Side Mount Modified (217-4239):1 ↔ #8-32 x 1.500 Star Drive Screw (276-4998):11
- Mate:675: Intake VersaFrame VersaPlanetary Side Mount Modified (217-4239):1 ↔ #8-32 Nylock Nut (275-1027):85
- Mate:676: Intake VersaFrame VersaPlanetary Side Mount Modified (217-4239):1 ↔ #8-32 Nylock Nut (275-1027):83
- Mate:677: Intake VersaFrame VersaPlanetary Side Mount Modified (217-4239):1 ↔ #8-32 Nylock Nut (275-1027):84
- Mate:678: Intake VersaFrame VersaPlanetary Side Mount Modified (217-4239):1 ↔ #8-32 x 0.500 Star Drive Screw (276-4992):6
- Mate:679: Intake VersaFrame VersaPlanetary Side Mount Modified (217-4239):1 ↔ #8-32 x 0.500 Star Drive Screw (276-4992):5
- Mate:680: Intake VersaFrame VersaPlanetary Side Mount Modified (217-4239):1 ↔ #8-32 x 0.500 Star Drive Screw (276-4992):5
- Mate:681: Intake VersaFrame VersaPlanetary Side Mount Modified (217-4239):1 ↔ #8-32 x 0.500 Star Drive Screw (276-4992):6
- Angle:275 (0 deg): Intake VersaFrame VersaPlanetary Side Mount Modified (217-4239):1 ↔ #8-32 x 0.500 Star Drive Screw (276-4992):5
- Angle:276 (0 deg): Intake VersaFrame VersaPlanetary Side Mount Modified (217-4239):1 ↔ #8-32 x 0.500 Star Drive Screw (276-4992):6
- Mate:682: Clamping Shaft Collar - 1_2 Hex ID (217-2737):1 ↔ Clamping Shaft Collar - 1_2 Hex ID (217-2737):12
- [Mate]: 1.00 Standoff (275-1016):3 ↔ #8-32 x 0.500 Star Drive Screw (276-4992):7
- [Mate]: Intake Motor Holder Using 1__16 Gray Tinted Polycarbonate Sheet (36 x 72) (217-6627):1 ↔ #8-32 x 0.500 Star Drive Screw (276-4992):8
- [Mate]: Intake Motor Holder Using 1__16 Gray Tinted Polycarbonate Sheet (36 x 72) (217-6627):2 ↔ #8-32 x 0.500 Star Drive Screw (276-4992):7
- [Mate]: Intake Motor Holder Using 1__16 Gray Tinted Polycarbonate Sheet (36 x 72) (217-6627):1 ↔ 1.00 Standoff (275-1016):3
- [Mate]: Intake Motor Holder Using 1__16 Gray Tinted Polycarbonate Sheet (36 x 72) (217-6627):2 ↔ #8-32 x 0.500 Star Drive Screw (276-4992):7
- [Mate]: Intake Motor Holder Using 1__16 Gray Tinted Polycarbonate Sheet (36 x 72) (217-6627):1 ↔ #8-32 x 0.500 Star Drive Screw (276-4992):8
- [Mate]: Intake Motor Holder Using 1__16 Gray Tinted Polycarbonate Sheet (36 x 72) (217-6627):2 ↔ 13.75mm (1_2 ThunderHex ID) x 1.125 OD x 0.313 WD (Flanged Bearing) (217-4006):11
- [Mate]: Intake Motor Holder Using 1__16 Gray Tinted Polycarbonate Sheet (36 x 72) (217-6627):1 ↔ 13.75mm (1_2 ThunderHex ID) x 1.125 OD x 0.313 WD (Flanged Bearing) (217-4006):12
- [Mate]: Intake Motor Holder Using 1__16 Gray Tinted Polycarbonate Sheet (36 x 72) (217-6627):2 ↔ 13.75mm (1_2 ThunderHex ID) x 1.125 OD x 0.313 WD (Flanged Bearing) (217-4006):11
- [Mate]: Intake Motor Holder Using 1__16 Gray Tinted Polycarbonate Sheet (36 x 72) (217-6627):1 ↔ 13.75mm (1_2 ThunderHex ID) x 1.125 OD x 0.313 WD (Flanged Bearing) (217-4006):12
- [Mate]: 1_2 Acetal Spacer - 1_2 Hex (217-2758):7 ↔ 1_4 Acetal Spacer - 1_2 Hex (217-2758):17
- [Mate]: 1_4 Acetal Spacer - 1_2 Hex (217-2758):17 ↔ 1_8 Acetal Spacer - 1_2 Hex (217-2758):3
- [Mate]: 1_2 Acetal Spacer - 1_2 Hex (217-2758):7 ↔ 1_4 Acetal Spacer - 1_2 Hex (217-2758):17
- [Mate]: 1_4 Acetal Spacer - 1_2 Hex (217-2758):17 ↔ 1_8 Acetal Spacer - 1_2 Hex (217-2758):3
- [Angle] (0 deg): 1_2 Acetal Spacer - 1_2 Hex (217-2758):7 ↔ 1_4 Acetal Spacer - 1_2 Hex (217-2758):17
- [Angle] (0 deg): 1_2 Acetal Spacer - 1_2 Hex (217-2758):7 ↔ 1_8 Acetal Spacer - 1_2 Hex (217-2758):3
- [Mate]: 13.75mm (1_2 ThunderHex ID) x 1.125 OD x 0.313 WD (Flanged Bearing) (217-4006):11 ↔ 1_8 Acetal Spacer - 1_2 Hex (217-2758):3
- [Mate]: 13.75mm (1_2 ThunderHex ID) x 1.125 OD x 0.313 WD (Flanged Bearing) (217-4006):11 ↔ 1_8 Acetal Spacer - 1_2 Hex (217-2758):3
- Mate:699: 1 x 1 x 0.040 x 14 Intake Pre-Drilled VersaFrame Aluminum Tube Stock Cut Modified (217-3426):1 ↔ Intake Motor Holder Using 1__16 Gray Tinted Polycarbonate Sheet (36 x 72) (217-6627):2
- Mate:700: 1 x 1 x 0.040 x 14 Intake Pre-Drilled VersaFrame Aluminum Tube Stock Cut Modified (217-3426):1 ↔ Intake Motor Holder Using 1__16 Gray Tinted Polycarbonate Sheet (36 x 72) (217-6627):2
- Mate:701: 1 x 1 x 0.040 x 14 Intake Pre-Drilled VersaFrame Aluminum Tube Stock Cut Modified (217-3426):1 ↔ Intake Motor Holder Using 1__16 Gray Tinted Polycarbonate Sheet (36 x 72) (217-6627):1
- Mate:702: 1 x 1 x 0.040 x 14 Intake Pre-Drilled VersaFrame Aluminum Tube Stock Cut Modified (217-3426):1 ↔ Intake Motor Holder Using 1__16 Gray Tinted Polycarbonate Sheet (36 x 72) (217-6627):1
- Mate:703: 1 x 1 x 0.040 x 14 Intake Pre-Drilled VersaFrame Aluminum Tube Stock Cut Modified (217-3426):1 ↔ Intake Motor Holder Using 1__16 Gray Tinted Polycarbonate Sheet (36 x 72) (217-6627):1
- Mate:704: 1 x 1 x 0.040 x 14 Intake Pre-Drilled VersaFrame Aluminum Tube Stock Cut Modified (217-3426):1 ↔ Intake Motor Holder Using 1__16 Gray Tinted Polycarbonate Sheet (36 x 72) (217-6627):2
- Mate:705: Intake Motor Holder Using 1__16 Gray Tinted Polycarbonate Sheet (36 x 72) (217-6627):2 ↔ #8-32 x 1.500 Star Drive Screw (276-4998):8
- Mate:706: Intake Motor Holder Using 1__16 Gray Tinted Polycarbonate Sheet (36 x 72) (217-6627):2 ↔ #8-32 x 1.500 Star Drive Screw (276-4998):6
- Mate:707: Intake Motor Holder Using 1__16 Gray Tinted Polycarbonate Sheet (36 x 72) (217-6627):2 ↔ #8-32 x 1.500 Star Drive Screw (276-4998):7
- Mate:708: Intake Motor Holder Using 1__16 Gray Tinted Polycarbonate Sheet (36 x 72) (217-6627):1 ↔ #8-32 Nylock Nut (275-1027):66
- Mate:709: Intake Motor Holder Using 1__16 Gray Tinted Polycarbonate Sheet (36 x 72) (217-6627):1 ↔ #8-32 Nylock Nut (275-1027):67
- Mate:710: Intake Motor Holder Using 1__16 Gray Tinted Polycarbonate Sheet (36 x 72) (217-6627):1 ↔ #8-32 Nylock Nut (275-1027):68
- Mate:711: Clamping Shaft Collar - 1_2 Hex ID (217-2737):1 ↔ 13.75mm (1_2 ThunderHex ID) x 1.125 OD x 0.313 WD (Flanged Bearing) (217-4006):12
- Angle:279 (0 deg): 1 x 1 x 0.040 x 14 Intake Pre-Drilled VersaFrame Aluminum Tube Stock Cut Modified (217-3426):1 ↔ 1.00 Standoff (275-1016):3
- Angle:280 (0 deg): 1 x 1 x 0.040 x 14 Intake Pre-Drilled VersaFrame Aluminum Tube Stock Cut Modified (217-3426):1 ↔ #8-32 x 0.500 Star Drive Screw (276-4992):7
- Angle:281 (0 deg): 1 x 1 x 0.040 x 14 Intake Pre-Drilled VersaFrame Aluminum Tube Stock Cut Modified (217-3426):1 ↔ #8-32 x 0.500 Star Drive Screw (276-4992):8
- Angle:282 (0 deg): 1 x 1 x 0.040 x 14 Intake Pre-Drilled VersaFrame Aluminum Tube Stock Cut Modified (217-3426):1 ↔ 13.75mm (1_2 ThunderHex ID) x 1.125 OD x 0.313 WD (Flanged Bearing) (217-4006):11
- Angle:283 (0 deg): 1 x 1 x 0.040 x 14 Intake Pre-Drilled VersaFrame Aluminum Tube Stock Cut Modified (217-3426):1 ↔ 13.75mm (1_2 ThunderHex ID) x 1.125 OD x 0.313 WD (Flanged Bearing) (217-4006):12
- Angle:284 (0 deg): 1 x 1 x 0.040 x 14 Intake Pre-Drilled VersaFrame Aluminum Tube Stock Cut Modified (217-3426):1 ↔ 1_2 Acetal Spacer - 1_2 Hex (217-2758):7
- Angle:285 (0 deg): 1 x 1 x 0.040 x 14 Intake Pre-Drilled VersaFrame Aluminum Tube Stock Cut Modified (217-3426):1 ↔ #8-32 x 2.000 Star Drive Screw (276-8015):70
- Angle:286 (0 deg): 1 x 1 x 0.040 x 14 Intake Pre-Drilled VersaFrame Aluminum Tube Stock Cut Modified (217-3426):1 ↔ #8-32 x 2.000 Star Drive Screw (276-8015):67
- Angle:287 (0 deg): 1 x 1 x 0.040 x 14 Intake Pre-Drilled VersaFrame Aluminum Tube Stock Cut Modified (217-3426):1 ↔ #8-32 x 2.000 Star Drive Screw (276-8015):71
- Angle:288 (0 deg): 1 x 1 x 0.040 x 14 Intake Pre-Drilled VersaFrame Aluminum Tube Stock Cut Modified (217-3426):1 ↔ #8-32 x 2.000 Star Drive Screw (276-8015):72
- Angle:289 (0 deg): 1 x 1 x 0.040 x 14 Intake Pre-Drilled VersaFrame Aluminum Tube Stock Cut Modified (217-3426):1 ↔ #8-32 x 2.000 Star Drive Screw (276-8015):68
- Angle:290 (0 deg): 1 x 1 x 0.040 x 14 Intake Pre-Drilled VersaFrame Aluminum Tube Stock Cut Modified (217-3426):1 ↔ #8-32 x 2.000 Star Drive Screw (276-8015):69
- Angle:291 (0 deg): 1 x 1 x 0.040 x 14 Intake Pre-Drilled VersaFrame Aluminum Tube Stock Cut Modified (217-3426):1 ↔ #8-32 x 2.000 Star Drive Screw (276-8015):24
- Angle:292 (0 deg): 1 x 1 x 0.040 x 14 Intake Pre-Drilled VersaFrame Aluminum Tube Stock Cut Modified (217-3426):1 ↔ #8-32 x 2.000 Star Drive Screw (276-8015):23
- Angle:293 (0 deg): 1 x 1 x 0.040 x 14 Intake Pre-Drilled VersaFrame Aluminum Tube Stock Cut Modified (217-3426):1 ↔ #8-32 x 2.000 Star Drive Screw (276-8015):22
- Angle:294 (0 deg): 1 x 1 x 0.040 x 14 Intake Pre-Drilled VersaFrame Aluminum Tube Stock Cut Modified (217-3426):1 ↔ #8-32 x 2.000 Star Drive Screw (276-8015):21
- Angle:295 (0 deg): 1 x 1 x 0.040 x 14 Intake Pre-Drilled VersaFrame Aluminum Tube Stock Cut Modified (217-3426):1 ↔ #8-32 x 2.000 Star Drive Screw (276-8015):20
- Angle:296 (0 deg): 1 x 1 x 0.040 x 14 Intake Pre-Drilled VersaFrame Aluminum Tube Stock Cut Modified (217-3426):1 ↔ #8-32 x 2.000 Star Drive Screw (276-8015):19
- Angle:297 (0 deg): 1 x 1 x 0.040 x 14 Intake Pre-Drilled VersaFrame Aluminum Tube Stock Cut Modified (217-3426):1 ↔ #8-32 x 2.000 Star Drive Screw (276-8015):48
- Angle:298 (0 deg): 1 x 1 x 0.040 x 14 Intake Pre-Drilled VersaFrame Aluminum Tube Stock Cut Modified (217-3426):1 ↔ #8-32 x 2.000 Star Drive Screw (276-8015):47
- Angle:299 (0 deg): 1 x 1 x 0.040 x 14 Intake Pre-Drilled VersaFrame Aluminum Tube Stock Cut Modified (217-3426):1 ↔ #8-32 x 2.000 Star Drive Screw (276-8015):46
- Angle:300 (0 deg): 1 x 1 x 0.040 x 14 Intake Pre-Drilled VersaFrame Aluminum Tube Stock Cut Modified (217-3426):1 ↔ #8-32 x 2.000 Star Drive Screw (276-8015):45
- Angle:301 (0 deg): 1 x 1 x 0.040 x 14 Intake Pre-Drilled VersaFrame Aluminum Tube Stock Cut Modified (217-3426):1 ↔ #8-32 x 2.000 Star Drive Screw (276-8015):44